# Autodesk Inventor assembly: Chassis
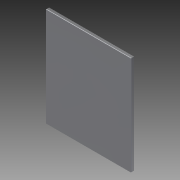
[picture p0: Inventor's stored thumbnail of the model, 180x180]
Saved by Autodesk Inventor 2013 (Build 170138000, 138)
## iProperties
Created: 2015-07-02
Part Number: Chassis
Document SubType Name: Assembly
Designer: Kyle
Mass: 87.1253 g
Surface Area: 574.146 cm^2
Volume: 56.6886 cm^3
Density: 1.53691 g/cm^3
Author: Kyle
## Documents named in this file (3)
- C:\Users\Kyle\Documents\Project documentation\Combat Robot\CAD\V1.0\Chassis.iam
- C:\Users\Kyle\Documents\Project documentation\Combat Robot\CAD\V1.0\Chassis_Poly.ipt
- C:\Users\Kyle\Documents\Project documentation\Combat Robot\CAD\V1.0\Chassis_Alu19.ipt
## Components (2 placed, 2 different names)
1. Chassis_Poly:1 — Mate:1, Flush:1, Flush:2
2. Chassis_Alu19:1 — Mate:1, Flush:1, Flush:2
## Relationships (3: Flush 2, Mate 1)
- Mate:1: Chassis_Poly:1 ↔ Chassis_Alu19:1
- Flush:1: Chassis_Poly:1 ↔ Chassis_Alu19:1
- Flush:2: Chassis_Poly:1 ↔ Chassis_Alu19:1
